# Autodesk Inventor assembly: top assembly
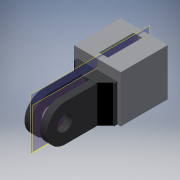
[picture p0: Inventor's stored thumbnail of the model, 180x180]
Saved by Autodesk Inventor 2016 (Build 200138000, 138)
## iProperties
Created: 2015-11-17
Part Number: top assembly
Document SubType Name: Assembly
Designer: Jesse Stevenson
Author: Jesse Stevenson
## Documents named in this file (3)
- C:\Users\Jesse Stevenson\Desktop\E-121-Design\light sensor mounts\top assembly.iam
- C:\Users\Jesse Stevenson\Desktop\E-121-Design\light sensor mounts\Light sensor shield 3.ipt
- C:\Users\Jesse Stevenson\Desktop\geared-extruder-drive-master\sw\gopro compat2.ipt
## Components (2 placed, 2 different names)
1. Light sensor shield 3:1 — Mate:1, Flush:1, Mate:2
2. gopro compat2:1 — Mate:1, Flush:1, Angle:1, Mate:3, Angle:2
## Relationships (7: Mate 4, Angle 2, Flush 1)
- Mate:1: Light sensor shield 3:1 ↔ gopro compat2:1
- Flush:1: Light sensor shield 3:1 ↔ gopro compat2:1
- Mate:2: Light sensor shield 3:1
- Angle:1 (0 deg): gopro compat2:1
- Mate:3: gopro compat2:1
- Angle:2 (0 deg): gopro compat2:1
- Mate:4
